# Autodesk Inventor assembly: _MK-1_Assembly
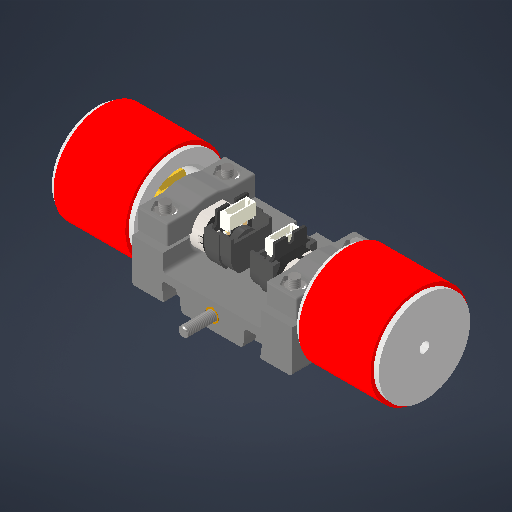
[picture p0: Inventor's stored thumbnail of the model, 512x512]
Saved by Autodesk Inventor 2026 (Build 300175000, 175)
## iProperties
Created: 2026-03-30
Part Number: _MK-1_Assembly
Document SubType Name: Assembly
Designer: zak
Author: zak
## Documents named in this file (11)
- C:\Users\vadim\GitHub\RoboCrew\Neo-Sumec\NeoSumec-MiniSumo-MECH\_MK-1_\_MK-1_Assembly.iam
- C:\Users\vadim\GitHub\RoboCrew\Neo-Sumec\NeoSumec-MiniSumo-MECH\_MK-1_\Models\3D_Print\MotorMountBottom.ipt
- C:\Users\vadim\GitHub\RoboCrew\Neo-Sumec\NeoSumec-MiniSumo-MECH\_MK-1_\Models\3rd-party_comp\Pololu Micro Metal Gearmotor 3D (STEP) Models\With Encoder, Side Connector\mmgm-cb-enc-side-con\mmgm-cb-enc-side-con\mmgm-cb-enc-side-con.ipt
- C:\Users\vadim\GitHub\RoboCrew\Neo-Sumec\NeoSumec-MiniSumo-MECH\_MK-1_\Models\3D_Print\MotorClamp.ipt
- C:\Users\vadim\GitHub\RoboCrew\Neo-Sumec\NeoSumec-MiniSumo-MECH\_MK-1_\Models\Metal\Wheel.ipt
- C:\Users\vadim\GitHub\RoboCrew\Neo-Sumec\NeoSumec-MiniSumo-MECH\_MK-1_\Models\Other technology\silicon bublebum.ipt
- C:\Users\vadim\GitHub\RoboCrew\Neo-Sumec\NeoSumec-MiniSumo-MECH\_MK-1_\Models\Metal\pipe.ipt
- C:\Users\vadim\GitHub\RoboCrew\Neo-Sumec\NeoSumec-MiniSumo-MECH\_MK-1_\SpojMat\DIN 934 - M3 x 0,5.ipt
- C:\Users\vadim\GitHub\RoboCrew\Neo-Sumec\NeoSumec-MiniSumo-MECH\_MK-1_\SpojMat\ISO 14581 - M3x20-4.8.ipt
- C:\Users\vadim\GitHub\RoboCrew\Neo-Sumec\NeoSumec-MiniSumo-MECH\_MK-1_\SpojMat\ISO 14581 - M3x16-4.8.ipt
- C:\Users\vadim\GitHub\RoboCrew\Neo-Sumec\NeoSumec-MiniSumo-MECH\_MK-1_\SpojMat\ISO 14580 M3x25-4.8.ipt
## Components (19 placed, 10 different names)
1. MotorMountBottom:1 — Stejný směr:1, Proti sobě:1, Stejný směr:2, Proti sobě:2, Proti sobě:4, Proti sobě:5, Proti sobě:7, Proti sobě:8, Proti sobě:13, Proti sobě:18, Proti sobě:19, Stejný směr:3, Proti sobě:20, Proti sobě:21, Proti sobě:35, Proti sobě:36, Proti sobě:37, Proti sobě:38, Proti sobě:39
2. mmgm-cb-enc-side-con:1 — Stejný směr:2, Proti sobě:2, Proti sobě:3, Proti sobě:9, Proti sobě:10
3. mmgm-cb-enc-side-con:2 — Stejný směr:1, Proti sobě:1, Proti sobě:6, Proti sobě:16, Proti sobě:17
4. MotorClamp:1 — Proti sobě:6, Proti sobě:7, Proti sobě:8, Proti sobě:23, Proti sobě:24, Proti sobě:29, Proti sobě:30, Proti sobě:31
5. MotorClamp:2 — Proti sobě:3, Proti sobě:4, Proti sobě:5, Proti sobě:25, Proti sobě:26, Proti sobě:27, Proti sobě:28, Proti sobě:32, Proti sobě:33
6. Wheel:1 — Proti sobě:14, Proti sobě:15, Proti sobě:16, Proti sobě:17, Proti sobě:18
7. Wheel:2 — Proti sobě:9, Proti sobě:10, Proti sobě:11, Proti sobě:12, Proti sobě:13
8. silicon bublebum:1 — Proti sobě:11, Proti sobě:12
9. silicon bublebum:2 — Proti sobě:14, Proti sobě:15
10. pipe:1 — Proti sobě:19, Stejný směr:3, Proti sobě:40, Proti sobě:41
11. DIN 934 - M3 x 0,5:1 — Proti sobě:29, Proti sobě:30, Proti sobě:31
12. DIN 934 - M3 x 0,5:2 — Proti sobě:28, Proti sobě:32, Proti sobě:33
13. DIN 934 - M3 x 0,5:3 — Proti sobě:25, Proti sobě:26, Proti sobě:27, Proti sobě:34
14. DIN 934 - M3 x 0,5:4 — Proti sobě:22, Proti sobě:23, Proti sobě:24
15. ISO 14581 - M3x20-4.8:1 — Proti sobě:34, Proti sobě:35
16. ISO 14581 - M3x20-4.8:2 — Proti sobě:20, Proti sobě:21, Proti sobě:22
17. ISO 14581 - M3x16-4.8:1 — Proti sobě:36, Proti sobě:37
18. ISO 14581 - M3x16-4.8:2 — Proti sobě:38, Proti sobě:39
19. ISO 14580 M3x25-4.8:1 — Proti sobě:40, Proti sobě:41
## Relationships (44: Mate 41, Flush 3)
- Stejný směr:1 [Flush] (-5 mm): MotorMountBottom:1 ↔ mmgm-cb-enc-side-con:2
- Proti sobě:1 [Mate]: MotorMountBottom:1 ↔ mmgm-cb-enc-side-con:2
- Stejný směr:2 [Flush] (-5 mm): MotorMountBottom:1 ↔ mmgm-cb-enc-side-con:1
- Proti sobě:2 [Mate]: MotorMountBottom:1 ↔ mmgm-cb-enc-side-con:1
- Proti sobě:3 [Mate]: mmgm-cb-enc-side-con:1 ↔ MotorClamp:2
- Proti sobě:4 [Mate]: MotorMountBottom:1 ↔ MotorClamp:2
- Proti sobě:5 [Mate]: MotorMountBottom:1 ↔ MotorClamp:2
- Proti sobě:6 [Mate]: mmgm-cb-enc-side-con:2 ↔ MotorClamp:1
- Proti sobě:7 [Mate]: MotorMountBottom:1 ↔ MotorClamp:1
- Proti sobě:8 [Mate]: MotorMountBottom:1 ↔ MotorClamp:1
- Proti sobě:9 [Mate]: mmgm-cb-enc-side-con:1 ↔ Wheel:2
- Proti sobě:10 [Mate] (0.1 mm): mmgm-cb-enc-side-con:1 ↔ Wheel:2
- Proti sobě:11 [Mate]: Wheel:2 ↔ silicon bublebum:1
- Proti sobě:12 [Mate]: Wheel:2 ↔ silicon bublebum:1
- Proti sobě:13 [Mate] (0.5 mm): MotorMountBottom:1 ↔ Wheel:2
- Proti sobě:14 [Mate]: Wheel:1 ↔ silicon bublebum:2
- Proti sobě:15 [Mate]: Wheel:1 ↔ silicon bublebum:2
- Proti sobě:16 [Mate]: mmgm-cb-enc-side-con:2 ↔ Wheel:1
- Proti sobě:17 [Mate] (0.25 mm): mmgm-cb-enc-side-con:2 ↔ Wheel:1
- Proti sobě:18 [Mate] (0.5 mm): MotorMountBottom:1 ↔ Wheel:1
- Proti sobě:19 [Mate]: MotorMountBottom:1 ↔ pipe:1
- Stejný směr:3 [Flush]: MotorMountBottom:1 ↔ pipe:1
- Proti sobě:20 [Mate]: MotorMountBottom:1 ↔ ISO 14581 - M3x20-4.8:2
- Proti sobě:21 [Mate]: MotorMountBottom:1 ↔ ISO 14581 - M3x20-4.8:2
- Proti sobě:22 [Mate]: DIN 934 - M3 x 0,5:4 ↔ ISO 14581 - M3x20-4.8:2
- Proti sobě:23 [Mate] (0.125 mm): MotorClamp:1 ↔ DIN 934 - M3 x 0,5:4
- Proti sobě:24 [Mate]: MotorClamp:1 ↔ DIN 934 - M3 x 0,5:4
- Proti sobě:25 [Mate] (0.125 mm): MotorClamp:2 ↔ DIN 934 - M3 x 0,5:3
- Proti sobě:26 [Mate]: MotorClamp:2 ↔ DIN 934 - M3 x 0,5:3
- Proti sobě:27 [Mate]: MotorClamp:2 ↔ DIN 934 - M3 x 0,5:3
- Proti sobě:28 [Mate]: MotorClamp:2 ↔ DIN 934 - M3 x 0,5:2
- Proti sobě:29 [Mate]: MotorClamp:1 ↔ DIN 934 - M3 x 0,5:1
- Proti sobě:30 [Mate] (0.125 mm): MotorClamp:1 ↔ DIN 934 - M3 x 0,5:1
- Proti sobě:31 [Mate]: MotorClamp:1 ↔ DIN 934 - M3 x 0,5:1
- Proti sobě:32 [Mate] (0.125 mm): MotorClamp:2 ↔ DIN 934 - M3 x 0,5:2
- Proti sobě:33 [Mate]: MotorClamp:2 ↔ DIN 934 - M3 x 0,5:2
- Proti sobě:34 [Mate]: DIN 934 - M3 x 0,5:3 ↔ ISO 14581 - M3x20-4.8:1
- Proti sobě:35 [Mate]: MotorMountBottom:1 ↔ ISO 14581 - M3x20-4.8:1
- Proti sobě:36 [Mate]: MotorMountBottom:1 ↔ ISO 14581 - M3x16-4.8:1
- Proti sobě:37 [Mate]: MotorMountBottom:1 ↔ ISO 14581 - M3x16-4.8:1
- Proti sobě:38 [Mate]: MotorMountBottom:1 ↔ ISO 14581 - M3x16-4.8:2
- Proti sobě:39 [Mate]: MotorMountBottom:1 ↔ ISO 14581 - M3x16-4.8:2
- Proti sobě:40 [Mate]: pipe:1 ↔ ISO 14580 M3x25-4.8:1
- Proti sobě:41 [Mate]: pipe:1 ↔ ISO 14580 M3x25-4.8:1
